# Autodesk Inventor assembly: !tower
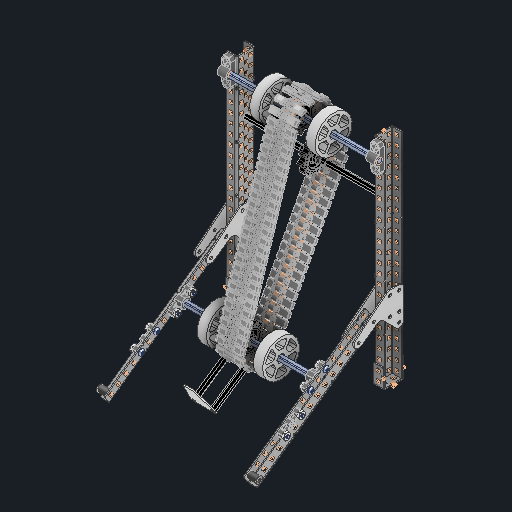
[picture p0: Inventor's stored thumbnail of the model, 512x512]
Saved by Autodesk Inventor 2025 (Build 290162000, 162)
## iProperties
Created: 2024-10-13
Part Number: !tower
Document SubType Name: Assembly
Designer: Averey Ku
Author: Averey Ku
## Documents named in this file (21)
- D:\vex_robotics_high_stakes\hardware\cad\bots\high_stakes_v2\tower\!tower.iam
- D:\vex_robotics_high_stakes\hardware\cad\bots\high_stakes_v2\tower\structure\!structure.iam
- D:\vex_robotics_high_stakes\hardware\cad\robpros_cad_lib\Motion\Shaft HS\Shaft HS\Shaft HS 7.5 in.ipt
- D:\vex_robotics_high_stakes\hardware\cad\robpros_cad_lib\Motion\Shaft HS\Shaft HS.ipt
- D:\vex_robotics_high_stakes\hardware\cad\robpros_cad_lib\Motion\Sprockets\9P Sprocket.iam
- D:\vex_robotics_high_stakes\hardware\cad\robpros_cad_lib\Motion\Sprockets\9P Sprocket\9P 12T Sprocket, No Insert.iam
- D:\vex_robotics_high_stakes\hardware\cad\robpros_cad_lib\Motion\Wheels\Flex Wheels\2.000 Flex Wheel\2.000 30A .500.ipt
- D:\vex_robotics_high_stakes\hardware\cad\robpros_cad_lib\Motion\Wheels\Flex Wheels\2.000 Flex Wheel.ipt
- D:\vex_robotics_high_stakes\hardware\cad\robpros_cad_lib\Motion\Shaft HS\Shaft HS\Shaft HS 8.5 in.ipt
- D:\vex_robotics_high_stakes\hardware\cad\bots\high_stakes_v2\tower\chain_path.ipt
- D:\vex_robotics_high_stakes\hardware\cad\robpros_cad_lib\Motion\Chain 9P\Tank Tread Traction Link.ipt
- D:\vex_robotics_high_stakes\hardware\cad\robpros_cad_lib\Motion\Chain 9P\Chain Attachment Link.ipt
- D:\vex_robotics_high_stakes\hardware\cad\robpros_cad_lib\Structure\Standoff\Standoff .25.ipt
- D:\vex_robotics_high_stakes\hardware\cad\robpros_cad_lib\Structure\Standoff.ipt
- D:\vex_robotics_high_stakes\hardware\cad\robpros_cad_lib\Structure\Standoff\Standoff 3.00.ipt
- D:\vex_robotics_high_stakes\hardware\cad\robpros_cad_lib\Motion\Spacers\Spacer Nylon .375 OD\NSpacer .375 OD x .125.ipt
- D:\vex_robotics_high_stakes\hardware\cad\robpros_cad_lib\Motion\Spacers\Spacer Nylon .375 OD.ipt
- D:\vex_robotics_high_stakes\hardware\cad\robpros_cad_lib\Motion\Spacers\Washer Steel\SWasher .375 OD x .031250.ipt
- D:\vex_robotics_high_stakes\hardware\cad\robpros_cad_lib\Motion\Spacers\Washer Steel.ipt
- D:\vex_robotics_high_stakes\hardware\cad\robpros_cad_lib\Structure\Standoff\Standoff 2.00.ipt
- D:\vex_robotics_high_stakes\hardware\cad\bots\high_stakes_v2\intake\custom_parts\hook_gusset.ipt
## Components (87 placed, 14 different names)
1. !structure:1 [sub-assembly] — Insert:1, Insert:2, Insert:5, Insert:11, Insert:17
2. Shaft HS 7.5 in:1 — Insert:1
3. 9P 12T Sprocket, No Insert:2 [sub-assembly] — Insert:2, Insert:3, Insert:4, Flush:1, Flush:3
4. 2.000 30A .500:1 — Insert:3
5. 2.000 30A .500:2 — Insert:4
6. Shaft HS 8.5 in:2 — Insert:5, Mate:1
7. 9P 12T Sprocket, No Insert:3 [sub-assembly] — Flush:1, Mate:1, Insert:6, Insert:7, Flush:2, Mate:3
8. 2.000 30A .500:3 — Insert:6
9. 2.000 30A .500:4 — Insert:7
10. 9P 12T Sprocket, No Insert:4 [sub-assembly] — Flush:2
11. chain_path:1 — Flush:3, Mate:4, Angle:1
12. Chain Attachment Link:1 — Insert:9, Mate:5
13. Standoff .25:1 — Insert:10, Insert:13
14. Standoff 3.00:2 — Insert:10, Insert:11
15. NSpacer .375 OD x .125:1 — Insert:12, Insert:13
16. SWasher .375 OD x .031250:1 — Insert:12
17. Standoff .25:3
18. Standoff 3.00:4 — Insert:17
19. NSpacer .375 OD x .125:2
20. SWasher .375 OD x .031250:2
21. Standoff 2.00:5 — Insert:19, Mate:7
22. Standoff 2.00:6 — Insert:18, Insert:21
23. Chain Attachment Link:2 — Insert:18, Insert:19, Insert:20, Mate:6
24. hook_gusset:1 — Insert:21, Mate:7
25. Tank Tread Traction Link:1 — Mate:3, Mate:4, Angle:1
26. Tank Tread Traction Link:2
27. Tank Tread Traction Link:3
28. Tank Tread Traction Link:4
29. Tank Tread Traction Link:5
30. Tank Tread Traction Link:6
31. Tank Tread Traction Link:7
32. Tank Tread Traction Link:8
33. Tank Tread Traction Link:9
34. Tank Tread Traction Link:10
35. Tank Tread Traction Link:11
36. Tank Tread Traction Link:12
37. Tank Tread Traction Link:13
38. Tank Tread Traction Link:14
39. Tank Tread Traction Link:15
40. Tank Tread Traction Link:16
41. Tank Tread Traction Link:17
42. Tank Tread Traction Link:18
43. Tank Tread Traction Link:19
44. Tank Tread Traction Link:20
45. Tank Tread Traction Link:21
46. Tank Tread Traction Link:22
47. Tank Tread Traction Link:23
48. Tank Tread Traction Link:24
49. Tank Tread Traction Link:25
50. Tank Tread Traction Link:26
51. Tank Tread Traction Link:27
52. Tank Tread Traction Link:28
53. Tank Tread Traction Link:29
54. Tank Tread Traction Link:30
55. Tank Tread Traction Link:31
56. Tank Tread Traction Link:32
57. Tank Tread Traction Link:33
58. Tank Tread Traction Link:34
59. Tank Tread Traction Link:35
60. Tank Tread Traction Link:36
61. Tank Tread Traction Link:37
62. Tank Tread Traction Link:38
63. Tank Tread Traction Link:39
64. Tank Tread Traction Link:40
65. Tank Tread Traction Link:41
66. Tank Tread Traction Link:42
67. Tank Tread Traction Link:43
68. Tank Tread Traction Link:44
69. Tank Tread Traction Link:45
70. Tank Tread Traction Link:46
71. Tank Tread Traction Link:47
72. Tank Tread Traction Link:48
73. Tank Tread Traction Link:49
74. Tank Tread Traction Link:50
75. Tank Tread Traction Link:51
76. Tank Tread Traction Link:52
77. Tank Tread Traction Link:53 — Insert:9, Mate:5
78. Tank Tread Traction Link:54
79. Tank Tread Traction Link:55
80. Tank Tread Traction Link:56
81. Tank Tread Traction Link:57
82. Tank Tread Traction Link:58
83. Tank Tread Traction Link:59
84. Tank Tread Traction Link:60 — Insert:20, Mate:6
85. Tank Tread Traction Link:61
86. Tank Tread Traction Link:62
87. Tank Tread Traction Link:63
## Component patterns: (63 elements, first: Tank Tread Traction Link:1)
## Relationships (30: Insert 20, Mate 6, Flush 3, Angle 1)
- Insert:1: !structure:1 ↔ Shaft HS 7.5 in:1
- Insert:2 (87.9094 mm): !structure:1 ↔ 9P 12T Sprocket, No Insert:2
- Insert:3 (25.4 mm): 9P 12T Sprocket, No Insert:2 ↔ 2.000 30A .500:1
- Insert:4 (25.4 mm): 9P 12T Sprocket, No Insert:2 ↔ 2.000 30A .500:2
- Insert:5: !structure:1 ↔ Shaft HS 8.5 in:2
- Flush:1: 9P 12T Sprocket, No Insert:2 ↔ 9P 12T Sprocket, No Insert:3
- Mate:1: Shaft HS 8.5 in:2 ↔ 9P 12T Sprocket, No Insert:3
- Insert:6 (25.4 mm): 9P 12T Sprocket, No Insert:3 ↔ 2.000 30A .500:3
- Insert:7 (25.4 mm): 9P 12T Sprocket, No Insert:3 ↔ 2.000 30A .500:4
- Flush:2: 9P 12T Sprocket, No Insert:3 ↔ 9P 12T Sprocket, No Insert:4
- Flush:3: 9P 12T Sprocket, No Insert:2 ↔ chain_path:1
- Mate:3: 9P 12T Sprocket, No Insert:3 ↔ Tank Tread Traction Link:1
- Mate:4: chain_path:1 ↔ Tank Tread Traction Link:1
- Angle:1 (-90 deg): chain_path:1 ↔ Tank Tread Traction Link:1
- Insert:9: Chain Attachment Link:1 ↔ Tank Tread Traction Link:53
- Mate:5: Chain Attachment Link:1 ↔ Tank Tread Traction Link:53
- Insert:10: Standoff .25:1 ↔ Standoff 3.00:2
- Insert:11: !structure:1 ↔ Standoff 3.00:2
- Insert:12: NSpacer .375 OD x .125:1 ↔ SWasher .375 OD x .031250:1
- Insert:13: Standoff .25:1 ↔ NSpacer .375 OD x .125:1
- [Insert]: Standoff .25:3 ↔ Standoff 3.00:4
- [Insert]: NSpacer .375 OD x .125:2 ↔ SWasher .375 OD x .031250:2
- [Insert]: Standoff .25:3 ↔ NSpacer .375 OD x .125:2
- Insert:17: !structure:1 ↔ Standoff 3.00:4
- Insert:18: Standoff 2.00:6 ↔ Chain Attachment Link:2
- Insert:19: Standoff 2.00:5 ↔ Chain Attachment Link:2
- Insert:20: Chain Attachment Link:2 ↔ Tank Tread Traction Link:60
- Mate:6: Chain Attachment Link:2 ↔ Tank Tread Traction Link:60
- Insert:21: Standoff 2.00:6 ↔ hook_gusset:1
- Mate:7: Standoff 2.00:5 ↔ hook_gusset:1
## Named parameters: d31_d27 = 0 mm, d32_d29 = 0 mm, d33_d30 = 0 mm
